# Autodesk Inventor assembly: GP-WSM010
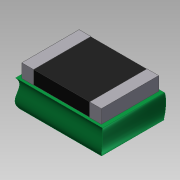
[picture p0: Inventor's stored thumbnail of the model, 180x180]
Saved by Autodesk Inventor 2011 (Build 150239000, 239)
## iProperties
Created: 2010-12-28
Part Number: GP-WSM010
Document SubType Name: Assembly
Designer: abbath
Mass: 0.0411691 g
Surface Area: 1.10238 cm^2
Volume: 0.0411691 cm^3
Density: 1 g/cm^3
Author: abbath
## Documents named in this file (3)
- D:\Abbath\Work\11.2\Сумматор light\КД\RSXX к сумматору\Установка элементов\GP-WSM010 установка.iam
- D:\Abbath\Work\11.2\Сумматор light\КД\RSXX к сумматору\Установка элементов\GP-WSM010.ipt
- D:\Abbath\Work\11.2\Сумматор light\КД\RSXX к сумматору\Установка элементов\GP-WSM010 плата.ipt
## Components (2 placed, 2 different names)
1. GP-WSM010:1 — Заподлицо:1
2. GP-WSM010 плата:1 — Заподлицо:1
## Relationships (1: Flush 1)
- Заподлицо:1 [Flush]: GP-WSM010:1 ↔ GP-WSM010 плата:1
